# Autodesk Inventor assembly: Non-Rotating Carousel Section Assembly
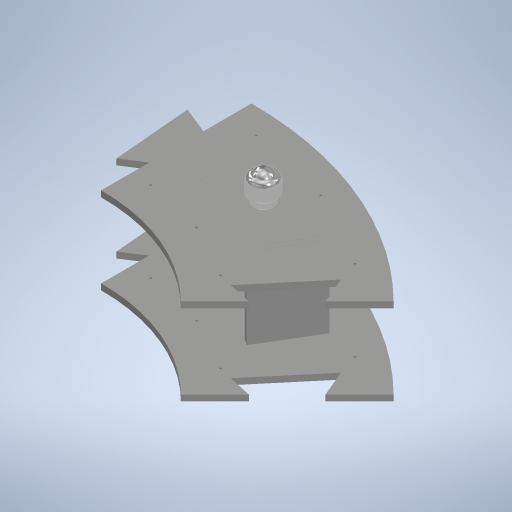
[picture p0: Inventor's stored thumbnail of the model, 512x512]
Saved by Autodesk Inventor 2023 (Build 270158000, 158)
## iProperties
Created: 2023-02-13
Part Number: Non-Rotating Carousel Section Assembly
Document SubType Name: Assembly
Designer: cheng
Author: cheng
## Documents named in this file (4)
- C:\Users\mihal\Desktop\4th Year Project\Final Assembly\Non-Rotating Carousel\Non-Rotating Carousel Section Assembly.iam
- C:\Users\mihal\Desktop\4th Year Project\Final Assembly\Non-Rotating Carousel\Base Plate Bottom v3.ipt
- C:\Users\mihal\Desktop\4th Year Project\Final Assembly\Non-Rotating Carousel\Base Plate Wall.ipt
- C:\Users\mihal\Desktop\4th Year Project\Final Assembly\Non-Rotating Carousel\WDS568-219-STEP-AP203\WDS568-219.ipt
## Components (5 placed, 3 different names)
1. Base Plate Bottom v3:1 — Mate:1, Flush:1, Mate:2, Flush:2, Mate:3, Mate:4
2. Base Plate Bottom v3:2 — Mate:5, Flush:3, Mate:6, Mate:7, Mate:8
3. Base Plate Wall:1 — Mate:1, Flush:1, Mate:2, Mate:5, Flush:3, Mate:6
4. Base Plate Wall:2 — Flush:2, Mate:3, Mate:4
5. WDS568-219:1 — Mate:7, Mate:8
## Relationships (11: Mate 8, Flush 3)
- Mate:1: Base Plate Bottom v3:1 ↔ Base Plate Wall:1
- Flush:1: Base Plate Bottom v3:1 ↔ Base Plate Wall:1
- Mate:2: Base Plate Bottom v3:1 ↔ Base Plate Wall:1
- Flush:2: Base Plate Bottom v3:1 ↔ Base Plate Wall:2
- Mate:3: Base Plate Bottom v3:1 ↔ Base Plate Wall:2
- Mate:4: Base Plate Bottom v3:1 ↔ Base Plate Wall:2
- Mate:5: Base Plate Bottom v3:2 ↔ Base Plate Wall:1
- Flush:3: Base Plate Bottom v3:2 ↔ Base Plate Wall:1
- Mate:6: Base Plate Bottom v3:2 ↔ Base Plate Wall:1
- Mate:7: Base Plate Bottom v3:2 ↔ WDS568-219:1
- Mate:8: Base Plate Bottom v3:2 ↔ WDS568-219:1
